# Autodesk Inventor assembly: 2307-0006-0028 bevel gear reverse mount
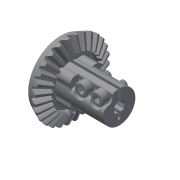
[picture p0: Inventor's stored thumbnail of the model, 180x180]
Saved by Autodesk Inventor 2018 (Build 220112000, 112)
## iProperties
Created: 2019-01-13
Part Number: 2307-0006-0028 bevel gear reverse mount
Document SubType Name: Assembly
Designer: ball
Author: ball
## Documents named in this file (3)
- C:\FTC\FTC8863CAD\GoBilda\2307 parts\2307-0006-0028 bevel gear reverse mount.iam
- C:\FTC\FTC8863CAD\GoBilda\2307 parts\2307-0006-0028.ipt
- C:\FTC\FTC8863CAD\GoBilda\1306 Parts\1306-0016-1006 assembly.ipt
## Components (2 placed, 2 different names)
1. 2307-0006-0028:1 — Mate:1, Mate:2, Mate:3
2. 1306-0016-1006 assembly:1 — Mate:1, Mate:2, Mate:3
## Relationships (3: Mate 3)
- Mate:1: 2307-0006-0028:1 ↔ 1306-0016-1006 assembly:1
- Mate:2: 2307-0006-0028:1 ↔ 1306-0016-1006 assembly:1
- Mate:3: 2307-0006-0028:1 ↔ 1306-0016-1006 assembly:1
